# Autodesk Inventor assembly: Assembly Rev D
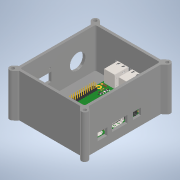
[picture p0: Inventor's stored thumbnail of the model, 180x180]
Saved by Autodesk Inventor 2021 (Build 250183000, 183)
## iProperties
Created: 2021-07-28
Part Number: Assembly Rev D
Document SubType Name: Assembly
Designer: cmzgt
Author: cmzgt
## Documents named in this file (4)
- D:\Projects\CAD-Designs\RPICase\Rev F\RPi Case Rev F.iam
- D:\Projects\CAD-Designs\RPICase\Rev F\References\RPi Model\Raspberry Pi 3.iam
- D:\Projects\CAD-Designs\RPICase\Rev F\Case Rev F.ipt
- D:\Projects\CAD-Designs\RPICase\Rev F\Case Cover Rev F.ipt
## Components (3 placed, 3 different names)
1. Case Rev F:1 — Mate:1, Mate:2, Flush:1
2. Raspberry Pi 3:1 [sub-assembly] — Mate:1, Mate:2
3. Case Cover Rev F:1 — Flush:1
## Relationships (3: Mate 2, Flush 1)
- Mate:1: Case Rev F:1 ↔ Raspberry Pi 3:1
- Mate:2: Case Rev F:1 ↔ Raspberry Pi 3:1
- Flush:1: Case Rev F:1 ↔ Case Cover Rev F:1
